# Autodesk Inventor assembly: Battery_Tray
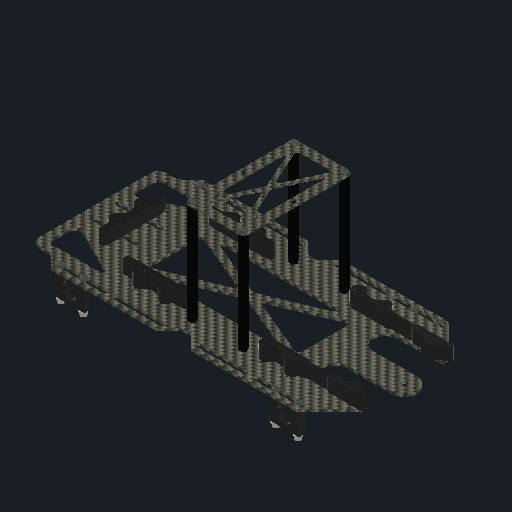
[picture p0: Inventor's stored thumbnail of the model, 512x512]
Saved by Autodesk Inventor 2025 (Build 290162010, 162A)
## iProperties
Created: 2023-12-07
Part Number: Battery_Tray
Document SubType Name: Assembly
Designer: dzw04
Mass: 130.423 g
Surface Area: 839.755 cm^2
Volume: 73.3709 cm^3
Density: 1.77759 g/cm^3
Author: dzw04
## Documents named in this file (10)
- C:\Users\dhrzw\OneDrive - Saxion\Sarax_Pack_And_Go\Workspaces\Workspace\SARAX\01. CAD\01. 3D_Drawing\02. Sub_Assemblies\Battery_Tray\Battery_Tray.iam
- C:\Users\dhrzw\OneDrive - Saxion\Sarax_Pack_And_Go\Workspaces\Workspace\SARAX\01. CAD\01. 3D_Drawing\02. Sub_Assemblies\Battery_Tray\02. Sub_Assemblies\Battery_Clip_R.iam
- C:\Users\dhrzw\OneDrive - Saxion\Sarax_Pack_And_Go\Workspaces\Workspace\SARAX\01. CAD\01. 3D_Drawing\02. Sub_Assemblies\Battery_Tray\02. Sub_Assemblies\Battery_Clip_L.iam
- C:\Users\dhrzw\OneDrive - Saxion\Sarax_Pack_And_Go\Workspaces\Workspace\SARAX\01. CAD\01. 3D_Drawing\02. Sub_Assemblies\Battery_Tray\02. Sub_Assemblies\Battery_Slide.iam
- C:\Users\dhrzw\OneDrive - Saxion\Sarax_Pack_And_Go\Workspaces\Workspace\SARAX\01. CAD\01. 3D_Drawing\02. Sub_Assemblies\Battery_Tray\01. Parts\Battery_Tray.ipt
- C:\Users\dhrzw\OneDrive - Saxion\Sarax_Pack_And_Go\Workspaces\Workspace\SARAX\01. CAD\01. 3D_Drawing\02. Sub_Assemblies\Battery_Tray\01. Parts\Standoff_Battery.ipt
- C:\Users\dhrzw\OneDrive - Saxion\Sarax_Pack_And_Go\Workspaces\Workspace\SARAX\01. CAD\01. 3D_Drawing\02. Sub_Assemblies\Battery_Tray\01. Parts\Battery_Top_Tray.ipt
- C:\Users\dhrzw\OneDrive - Saxion\Sarax_Pack_And_Go\Workspaces\Workspace\SARAX\01. CAD\01. 3D_Drawing\02. Sub_Assemblies\Battery_Tray\02. Sub_Assemblies\12mm_Tube_Connector.iam
- C:\Users\dhrzw\OneDrive - Saxion\Sarax_Pack_And_Go\Workspaces\Workspace\SARAX\01. CAD\01. 3D_Drawing\01. Parts\en-US\ISO 7380-1\ISO 7380-1 - M3 x 8.ipt
- C:\Users\dhrzw\OneDrive - Saxion\Sarax_Pack_And_Go\Workspaces\Workspace\SARAX\01. CAD\01. 3D_Drawing\Parameters.xlsx
## Components (23 placed, 8 different names)
1. Battery_Tray:1 — Mate:1, Mate:2, Mate:3, Mate:4, Mate:5, Mate:8, Flush:4, Flush:5, Mate:11, Mate:12, Mate:13, Mate:14, Mate:15, Mate:16, Mate:17, Mate:18, Mate:22, Mate:23, Flush:16, Flush:17, Insert:1, Insert:2, Insert:3, Insert:4
2. Battery_Clip_R:1 [sub-assembly] — Mate:1, Flush:2, Mate:6, Mate:10
3. Battery_Clip_L:1 [sub-assembly] — Mate:2, Flush:2, Mate:6, Flush:3, Mate:8, Mate:9
4. Battery_Slide:1 [sub-assembly] — Mate:4, Flush:4, Mate:9
5. Battery_Slide:2 [sub-assembly] — Mate:3, Flush:1, Mate:7, Flush:3
6. Battery_Slide:3 [sub-assembly] — Mate:5, Flush:1, Mate:7, Mate:10, Flush:5
7. Standoff_Battery:1 — Mate:12, Mate:17, Flush:7, Mate:21
8. Standoff_Battery:2 — Mate:11, Mate:18, Flush:7
9. Standoff_Battery:3 — Mate:13, Mate:16, Flush:6
10. Standoff_Battery:4 — Mate:14, Mate:15, Flush:6, Mate:19, Mate:20
11. Battery_Top_Tray:1 — Mate:19, Mate:20, Mate:21, Insert:5, Insert:6, Insert:7, Insert:8
12. 12mm_Tube_Connector:1 [sub-assembly] — Flush:10, Flush:11, Mate:22, Flush:12, Flush:14, Flush:17
13. 12mm_Tube_Connector:2 [sub-assembly] — Flush:10, Flush:11, Flush:13, Flush:14, Flush:15, Flush:16
14. 12mm_Tube_Connector:3 [sub-assembly] — Flush:8, Flush:9, Flush:13, Flush:15
15. 12mm_Tube_Connector:4 [sub-assembly] — Flush:8, Flush:9, Mate:23, Flush:12
16. ISO 7380-1 M3 x 8:1 — Insert:1
17. ISO 7380-1 M3 x 8:2 — Insert:2
18. ISO 7380-1 M3 x 8:3 — Insert:3
19. ISO 7380-1 M3 x 8:4 — Insert:4
20. ISO 7380-1 M3 x 8:5 — Insert:5
21. ISO 7380-1 M3 x 8:6 — Insert:6
22. ISO 7380-1 M3 x 8:7 — Insert:7
23. ISO 7380-1 M3 x 8:8 — Insert:8
## Relationships (48: Mate 23, Flush 17, Insert 8)
- Mate:1: Battery_Tray:1 ↔ Battery_Clip_R:1
- Mate:2: Battery_Tray:1 ↔ Battery_Clip_L:1
- Mate:3: Battery_Tray:1 ↔ Battery_Slide:2
- Mate:4: Battery_Tray:1 ↔ Battery_Slide:1
- Mate:5: Battery_Tray:1 ↔ Battery_Slide:3
- Flush:1: Battery_Slide:2 ↔ Battery_Slide:3
- Flush:2: Battery_Clip_R:1 ↔ Battery_Clip_L:1
- Mate:6 (62 mm): Battery_Clip_R:1 ↔ Battery_Clip_L:1
- Mate:7 (62 mm): Battery_Slide:2 ↔ Battery_Slide:3
- Flush:3: Battery_Clip_L:1 ↔ Battery_Slide:2
- Mate:8 (-29 mm): Battery_Tray:1 ↔ Battery_Clip_L:1
- Flush:4 (35 mm): Battery_Tray:1 ↔ Battery_Slide:1
- Mate:9 (200 mm): Battery_Clip_L:1 ↔ Battery_Slide:1
- Mate:10 (125 mm): Battery_Clip_R:1 ↔ Battery_Slide:3
- Flush:5 (57.5 mm): Battery_Tray:1 ↔ Battery_Slide:3
- Mate:11: Battery_Tray:1 ↔ Standoff_Battery:2
- Mate:12: Battery_Tray:1 ↔ Standoff_Battery:1
- Mate:13: Battery_Tray:1 ↔ Standoff_Battery:3
- Mate:14: Battery_Tray:1 ↔ Standoff_Battery:4
- Mate:15: Battery_Tray:1 ↔ Standoff_Battery:4
- Mate:16: Battery_Tray:1 ↔ Standoff_Battery:3
- Mate:17: Battery_Tray:1 ↔ Standoff_Battery:1
- Mate:18: Battery_Tray:1 ↔ Standoff_Battery:2
- Flush:6: Standoff_Battery:3 ↔ Standoff_Battery:4
- Flush:7: Standoff_Battery:1 ↔ Standoff_Battery:2
- Mate:19: Standoff_Battery:4 ↔ Battery_Top_Tray:1
- Mate:20: Standoff_Battery:4 ↔ Battery_Top_Tray:1
- Mate:21: Standoff_Battery:1 ↔ Battery_Top_Tray:1
- Flush:8: 12mm_Tube_Connector:3 ↔ 12mm_Tube_Connector:4
- Flush:9: 12mm_Tube_Connector:3 ↔ 12mm_Tube_Connector:4
- Flush:10: 12mm_Tube_Connector:1 ↔ 12mm_Tube_Connector:2
- Flush:11: 12mm_Tube_Connector:1 ↔ 12mm_Tube_Connector:2
- Mate:22: Battery_Tray:1 ↔ 12mm_Tube_Connector:1
- Mate:23: Battery_Tray:1 ↔ 12mm_Tube_Connector:4
- Flush:12: 12mm_Tube_Connector:1 ↔ 12mm_Tube_Connector:4
- Flush:13: 12mm_Tube_Connector:2 ↔ 12mm_Tube_Connector:3
- Flush:14 (-170 mm): 12mm_Tube_Connector:1 ↔ 12mm_Tube_Connector:2
- Flush:15 (110 mm): 12mm_Tube_Connector:2 ↔ 12mm_Tube_Connector:3
- Flush:16 (2.5 mm): Battery_Tray:1 ↔ 12mm_Tube_Connector:2
- Flush:17 (25 mm): Battery_Tray:1 ↔ 12mm_Tube_Connector:1
- Insert:1: Battery_Tray:1 ↔ ISO 7380-1 M3 x 8:1
- Insert:2: Battery_Tray:1 ↔ ISO 7380-1 M3 x 8:2
- Insert:3: Battery_Tray:1 ↔ ISO 7380-1 M3 x 8:3
- Insert:4: Battery_Tray:1 ↔ ISO 7380-1 M3 x 8:4
- Insert:5: Battery_Top_Tray:1 ↔ ISO 7380-1 M3 x 8:5
- Insert:6: Battery_Top_Tray:1 ↔ ISO 7380-1 M3 x 8:6
- Insert:7: Battery_Top_Tray:1 ↔ ISO 7380-1 M3 x 8:7
- Insert:8: Battery_Top_Tray:1 ↔ ISO 7380-1 M3 x 8:8
## Named parameters: Width = 62 mm, Length = 200 mm, BatteryWidth = 62 mm, BatteryLength = 200 mm, BatteryHeight = 76 mm, NumberOfArms = 4, RotorToRotor = 900 mm, MountToMotorCenter = 0 mm, ArmPosition = 5 deg, ThicknessBodyCenterPlate = 2 mm, ThicknessBodyOuterPlate = 2 mm, ThicknessLegLoadpipePlate = 2 mm, ThicknessBatteryTray = 2 mm, ThicknessBatteryTopTray = 1 mm, LoadpipeLength = 450 mm, NumberOfBatterys = 2, LandingGearHeight = 400 mm, LandingGearStabilityBar = 525 mm, LandingGearRod = 390 mm, StartAngleArm = 45 deg, MotorMountCenter = 71.5 mm
